# Autodesk Inventor assembly: THREAD CLAMP SETUP
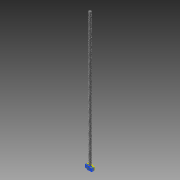
[picture p0: Inventor's stored thumbnail of the model, 180x180]
Saved by Autodesk Inventor 2013 (Build 170138000, 138)
## iProperties
Created: 2013-12-04
Part Number: THREAD CLAMP SETUP
Document SubType Name: Assembly
Designer: employee
Author: employee
## Documents named in this file (3)
- C:\Users\employee\Desktop\ConceptFORGE\ConceptFORGE\LISA Simpson\INVENTOR FILES\THREAD CLAMP SETUP.iam
- C:\Users\employee\Desktop\ConceptFORGE\ConceptFORGE\LISA Simpson\INVENTOR FILES\7_16 TORQSPLINE.ipt
- C:\Users\employee\Desktop\ConceptFORGE\ConceptFORGE\LISA Simpson\INVENTOR FILES\_THREAD CLAMP.ipt
## Components (3 placed, 2 different names)
1. _THREAD CLAMP:1
2. _THREAD CLAMP:2
3. 7_16 TORQSPLINE:1
## Relationships (6: Mate 3, Flush 2, Angle 1)
- [Flush]: _THREAD CLAMP:1 ↔ _THREAD CLAMP:2
- [Mate]: _THREAD CLAMP:1 ↔ _THREAD CLAMP:2
- [Mate]: _THREAD CLAMP:2
- [Angle] (0 deg): _THREAD CLAMP:1 ↔ _THREAD CLAMP:2
- [Flush]: _THREAD CLAMP:1 ↔ 7_16 TORQSPLINE:1
- [Mate]: _THREAD CLAMP:1 ↔ 7_16 TORQSPLINE:1
